# Autodesk Inventor assembly: 机械臂
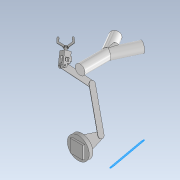
[picture p0: Inventor's stored thumbnail of the model, 180x180]
Saved by Autodesk Inventor 2022.5 (Build 265521000, 521)
## iProperties
Created: 2024-11-12
Part Number: 机械臂
Document SubType Name: Assembly
Designer: Gagouking
Author: Gagouking
## Documents named in this file (9)
- D:\Documents\好玩的\水下机器人\机械臂.iam
- D:\Documents\好玩的\水下机器人\底座.ipt
- D:\Documents\好玩的\水下机器人\大yaw.ipt
- D:\Documents\好玩的\水下机器人\大臂01.ipt
- D:\Documents\好玩的\水下机器人\小臂01.ipt
- D:\Documents\好玩的\水下机器人\合页01.ipt
- D:\Documents\好玩的\水下机器人\珊瑚.ipt
- D:\Documents\好玩的\水下机器人\夹爪连接件.ipt
- D:\Documents\好玩的\水下机器人\夹爪01.ipt
## Components (9 placed, 8 different names)
1. 底座:1 — 配合:1, 配合:2
2. 大yaw:1 — 配合:1, 配合:2, 配合:3, 配合:5
3. 大臂01:1 — 配合:3, 配合:4, 配合:5, 配合:6
4. 小臂01:1 — 配合:4, 配合:6, 配合:7, 配合:8
5. 合页01:1 — 配合:7, 配合:8, 配合:9, 配合:10
6. 珊瑚:1
7. 夹爪连接件:1 — 配合:9, 配合:10, 配合:11, 配合:12, 配合:13, 配合:14
8. 夹爪01:1 — 配合:11, 配合:12
9. 夹爪01:2 — 配合:13, 配合:14
## Relationships (14: Mate 14)
- 配合:1 [Mate]: 底座:1 ↔ 大yaw:1
- 配合:2 [Mate]: 底座:1 ↔ 大yaw:1
- 配合:3 [Mate]: 大yaw:1 ↔ 大臂01:1
- 配合:4 [Mate]: 大臂01:1 ↔ 小臂01:1
- 配合:5 [Mate]: 大yaw:1 ↔ 大臂01:1
- 配合:6 [Mate]: 大臂01:1 ↔ 小臂01:1
- 配合:7 [Mate]: 小臂01:1 ↔ 合页01:1
- 配合:8 [Mate]: 小臂01:1 ↔ 合页01:1
- 配合:9 [Mate]: 合页01:1 ↔ 夹爪连接件:1
- 配合:10 [Mate]: 合页01:1 ↔ 夹爪连接件:1
- 配合:11 [Mate]: 夹爪连接件:1 ↔ 夹爪01:1
- 配合:12 [Mate]: 夹爪连接件:1 ↔ 夹爪01:1
- 配合:13 [Mate]: 夹爪连接件:1 ↔ 夹爪01:2
- 配合:14 [Mate]: 夹爪连接件:1 ↔ 夹爪01:2
